# Autodesk Inventor assembly: s-assy-outer
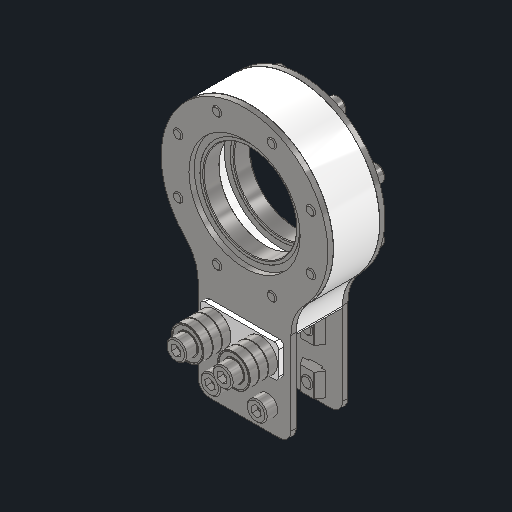
[picture p0: Inventor's stored thumbnail of the model, 512x512]
Saved by Autodesk Inventor 2022 (Build 260153000, 153)
## iProperties
Created: 2021-10-17
Part Number: s-assy-outer
Document SubType Name: Assembly
Designer: Yuta Kage
Author: Yuta Kage
## Documents named in this file (11)
- C:\Users\yuta0\Documents\GitHub\catchrobo_hardware\assy-scara\s-assy-outer.iam
- C:\Users\yuta0\Documents\GitHub\catchrobo_hardware\assy-scara\scara-base15.ipt
- C:\Users\yuta0\Documents\GitHub\catchrobo_hardware\assy-scara\CB4-25.ipt
- C:\Users\yuta0\Documents\GitHub\catchrobo_hardware\assy-scara\scara-plate9.ipt
- C:\Users\yuta0\Documents\GitHub\catchrobo_hardware\assy-scara\CB5-8.ipt
- C:\Users\yuta0\Documents\GitHub\catchrobo_hardware\assy-scara\scara-plate8.ipt
- C:\Users\yuta0\Documents\GitHub\catchrobo_hardware\assy-scara\MR148ZZ.ipt
- C:\Users\yuta0\Documents\GitHub\catchrobo_hardware\assy-scara\HNTT5-5.ipt
- C:\Users\yuta0\Documents\GitHub\catchrobo_hardware\assy-scara\B6808ZZ.ipt
- C:\Users\yuta0\Documents\GitHub\catchrobo_hardware\assy-scara\scara-base8.ipt
- C:\Users\yuta0\Documents\GitHub\catchrobo_hardware\assy-scara\CB5-22.ipt
## Components (38 placed, 10 different names)
1. scara-base15:1 — メイト:1, メイト:2, メイト:3, メイト:4, メイト:5, メイト:6, メイト:14, メイト:15, メイト:25
2. scara-plate9:1 — メイト:4, メイト:5, メイト:6, メイト:11, メイト:12, メイト:13, メイト:19, 角度:1, フラッシュ:2, メイト:22
3. scara-plate8:1 — メイト:1, メイト:2, メイト:3, メイト:7, メイト:8, メイト:9, メイト:10, メイト:17, メイト:26
4. B6808ZZ:2 — メイト:14, メイト:15
5. scara-base8:1 — メイト:20, メイト:21, メイト:22, メイト:23, メイト:24
6. B6808ZZ:3 — メイト:25, メイト:26
7. CB4-25:1 — メイト:7, メイト:8
8. CB4-25:2
9. CB4-25:3
10. CB4-25:4
11. CB4-25:5
12. CB4-25:6
13. CB4-25:7
14. CB4-25:8
15. CB5-8:2 — メイト:11, メイト:12, メイト:18
16. CB5-8:1 — メイト:9, メイト:10, メイト:16
17. HNTT5-5:2 — メイト:18, メイト:19, フラッシュ:1, 角度:1
18. HNTT5-5:1 — メイト:16, メイト:17, フラッシュ:1
19. CB5-8:3
20. CB5-8:4
21. HNTT5-5:3
22. HNTT5-5:6
23. CB5-8:5
24. CB5-8:6
25. HNTT5-5:4
26. HNTT5-5:7
27. CB5-8:7
28. CB5-8:8
29. HNTT5-5:5
30. HNTT5-5:8
31. MR148ZZ:1 — メイト:13
32. MR148ZZ:2 — メイト:20
33. MR148ZZ:3
34. MR148ZZ:4
35. MR148ZZ:5 — フラッシュ:2, メイト:21
36. MR148ZZ:6
37. CB5-22:1 — メイト:23, メイト:24
38. CB5-22:2
## Component patterns: (8 elements, first: CB4-25:1), (4 elements, first: CB5-8:2 + CB5-8:1 + HNTT5-5:2 + HNTT5-5:1), (6 elements, first: MR148ZZ:1), (2 elements, first: CB5-22:1)
## Relationships (29: Mate 26, Flush 2, Angle 1)
- メイト:1 [Mate]: scara-base15:1 ↔ scara-plate8:1
- メイト:2 [Mate]: scara-base15:1 ↔ scara-plate8:1
- メイト:3 [Mate]: scara-base15:1 ↔ scara-plate8:1
- メイト:4 [Mate]: scara-base15:1 ↔ scara-plate9:1
- メイト:5 [Mate]: scara-base15:1 ↔ scara-plate9:1
- メイト:6 [Mate]: scara-base15:1 ↔ scara-plate9:1
- メイト:7 [Mate]: scara-plate8:1 ↔ CB4-25:1
- メイト:8 [Mate]: scara-plate8:1 ↔ CB4-25:1
- メイト:9 [Mate]: scara-plate8:1 ↔ CB5-8:1
- メイト:10 [Mate]: scara-plate8:1 ↔ CB5-8:1
- メイト:11 [Mate]: scara-plate9:1 ↔ CB5-8:2
- メイト:12 [Mate]: scara-plate9:1 ↔ CB5-8:2
- メイト:13 [Mate]: scara-plate9:1 ↔ MR148ZZ:1
- メイト:14 [Mate]: scara-base15:1 ↔ B6808ZZ:2
- メイト:15 [Mate]: scara-base15:1 ↔ B6808ZZ:2
- メイト:16 [Mate]: CB5-8:1 ↔ HNTT5-5:1
- メイト:17 [Mate] (2 mm): scara-plate8:1 ↔ HNTT5-5:1
- メイト:18 [Mate]: CB5-8:2 ↔ HNTT5-5:2
- メイト:19 [Mate] (2 mm): scara-plate9:1 ↔ HNTT5-5:2
- フラッシュ:1 [Flush]: HNTT5-5:2 ↔ HNTT5-5:1
- 角度:1 [Angle] (0 deg): scara-plate9:1 ↔ HNTT5-5:2
- フラッシュ:2 [Flush] (-14.7 mm): scara-plate9:1 ↔ MR148ZZ:5
- メイト:20 [Mate]: scara-base8:1 ↔ MR148ZZ:2
- メイト:21 [Mate]: scara-base8:1 ↔ MR148ZZ:5
- メイト:22 [Mate]: scara-plate9:1 ↔ scara-base8:1
- メイト:23 [Mate]: scara-base8:1 ↔ CB5-22:1
- メイト:24 [Mate]: scara-base8:1 ↔ CB5-22:1
- メイト:25 [Mate]: scara-base15:1 ↔ B6808ZZ:3
- メイト:26 [Mate]: scara-plate8:1 ↔ B6808ZZ:3
